# Autodesk Inventor assembly: FrameAssembly
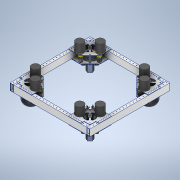
[picture p0: Inventor's stored thumbnail of the model, 180x180]
Saved by Autodesk Inventor 2020 (Build 240168000, 168)
## iProperties
Created: 2019-06-03
Part Number: FrameAssembly
Document SubType Name: Assembly
Designer: Connor
Author: Connor
## Documents named in this file (4)
- C:\Users\Connor\Documents\GrabCAD\2019 Robot\Swerve\TorqyoDrift\FrameAssembly.iam
- C:\Users\Connor\Documents\GrabCAD\2019 Robot\Swerve\TorqyoDrift\22in2x1Extrusion.ipt
- C:\Users\Connor\Documents\GrabCAD\2019 Robot\Swerve\TorqyoDrift\24in2x1Extrusion.ipt
- C:\Users\Connor\Documents\GrabCAD\2019 Robot\Swerve\TorqyoDrift\TestAssembly.iam
## Components (8 placed, 3 different names)
1. 22in2x1Extrusion:1 — Mate:1, Flush:1, Flush:2, Flush:7, Flush:11
2. 24in2x1Extrusion:1 — Mate:1, Flush:1, Flush:2, Mate:2, Flush:3, Flush:4, Mate:4, Flush:8, Mate:5, Flush:9
3. 22in2x1Extrusion:2 — Mate:2, Flush:3, Flush:4, Mate:3, Flush:5, Flush:6, Flush:10, Flush:13
4. 24in2x1Extrusion:2 — Mate:3, Flush:5, Flush:6, Mate:6, Flush:12, Mate:7, Flush:14
5. TestAssembly:1 [sub-assembly] — Mate:4, Flush:7, Flush:8
6. TestAssembly:2 [sub-assembly] — Mate:6, Flush:11, Flush:12
7. TestAssembly:3 [sub-assembly] — Mate:7, Flush:13, Flush:14
8. TestAssembly:4 [sub-assembly] — Mate:5, Flush:9, Flush:10
## Relationships (21: Flush 14, Mate 7)
- Mate:1: 22in2x1Extrusion:1 ↔ 24in2x1Extrusion:1
- Flush:1: 22in2x1Extrusion:1 ↔ 24in2x1Extrusion:1
- Flush:2: 22in2x1Extrusion:1 ↔ 24in2x1Extrusion:1
- Mate:2: 24in2x1Extrusion:1 ↔ 22in2x1Extrusion:2
- Flush:3: 24in2x1Extrusion:1 ↔ 22in2x1Extrusion:2
- Flush:4: 24in2x1Extrusion:1 ↔ 22in2x1Extrusion:2
- Mate:3: 22in2x1Extrusion:2 ↔ 24in2x1Extrusion:2
- Flush:5: 22in2x1Extrusion:2 ↔ 24in2x1Extrusion:2
- Flush:6: 22in2x1Extrusion:2 ↔ 24in2x1Extrusion:2
- Mate:4: 24in2x1Extrusion:1 ↔ TestAssembly:1
- Flush:7: 22in2x1Extrusion:1 ↔ TestAssembly:1
- Flush:8: 24in2x1Extrusion:1 ↔ TestAssembly:1
- Mate:5: 24in2x1Extrusion:1 ↔ TestAssembly:4
- Flush:9: 24in2x1Extrusion:1 ↔ TestAssembly:4
- Flush:10: 22in2x1Extrusion:2 ↔ TestAssembly:4
- Mate:6: 24in2x1Extrusion:2 ↔ TestAssembly:2
- Flush:11: 22in2x1Extrusion:1 ↔ TestAssembly:2
- Flush:12: 24in2x1Extrusion:2 ↔ TestAssembly:2
- Mate:7: 24in2x1Extrusion:2 ↔ TestAssembly:3
- Flush:13: 22in2x1Extrusion:2 ↔ TestAssembly:3
- Flush:14: 24in2x1Extrusion:2 ↔ TestAssembly:3
